(part 1 of 2)
# Autodesk Inventor assembly: Armature
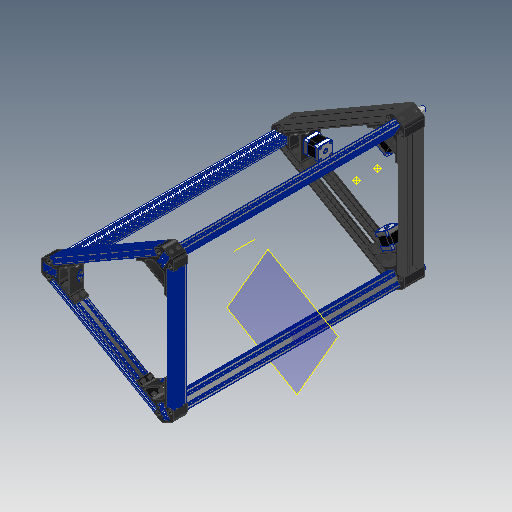
[picture p0: Inventor's stored thumbnail of the model, 512x512]
Saved by Autodesk Inventor 2017 (Build 210142000, 142)
## iProperties
Company: FABLAB Frenchmakers
Part Number: Armature
Material: Générique
Document SubType Name: Assembly
Designer: FABLAB Frenchmakers
Mass: 6567.24 g
Surface Area: 18690.5 cm^2
Volume: 2361.97 cm^3
Density: 2.78041 g/cm^3
Project: 1420 Vauban 3D XL
Stock Number: 1420-01-00
## Documents named in this file (13)
- W:\Professionnel\Conception FABLAB\1420-Vauban 3D XL\1420-01 Armature\1420-01-00 Armature.iam
- W:\Professionnel\Conception FABLAB\1420-Vauban 3D XL\1420-01 Armature\1420-01-14 Coins inferieur.iam
- W:\Professionnel\Conception FABLAB\1420-Vauban 3D XL\1420-01 Armature\1420-01-01 Profile vertical 20x40x750.ipt
- W:\Professionnel\Conception FABLAB\1420-Vauban 3D XL\1420-01 Armature\1420-01-15 Coins superieur.iam
- W:\Professionnel\Conception FABLAB\1420-Vauban 3D XL\1420-01 Armature\1420-01-03 Profile horizontal 20x20x360.ipt
- W:\Professionnel\Conception FABLAB\1420-Vauban 3D XL\1420-01 Armature\1420-01-02 Profile horizontal 20x40x360.ipt
- W:\Professionnel\Conception FABLAB\1420-Vauban 3D XL\1420-90 Centre de contenu\fr-FR\ANSI B18.3.1M(1)\ANSI B18.3.1M - M5x0,8 x 12(2).ipt
- W:\Professionnel\Conception FABLAB\1420-Vauban 3D XL\1420-90 Centre de contenu\fr-FR\DIN 125-1  A\DIN 125 - A 5,3.ipt
- W:\Professionnel\Conception FABLAB\1420-Vauban 3D XL\1420-01 Armature\1420-01-13 Noix M5.ipt
- W:\Professionnel\Conception FABLAB\1420-Vauban 3D XL\1420-90 Centre de contenu\fr-FR\DIN 7991(2)\DIN 7991 - M4x10.ipt
- W:\Professionnel\Conception FABLAB\1420-Vauban 3D XL\1420-01 Armature\1420-01-12 Noix M4.ipt
- W:\Professionnel\Conception FABLAB\1420-Vauban 3D XL\1420-01 Armature\1420-01-09 Pied.ipt
- W:\Professionnel\Conception FABLAB\1420-Vauban 3D XL\1420-90 Centre de contenu\fr-FR\ANSI B18.3.1M(1)\ANSI B18.3.1M - M5x0,8 x 25(2).ipt
## Components (192 placed, 12 different names)
1. 1420-01-09 Pied:1 — Affleurement:196, Placage:246, Placage:247, Placage:250, Placage:251
2. 1420-01-09 Pied:2 — Affleurement:196, Affleurement:197, Placage:249, Placage:253
3. 1420-01-09 Pied:3 — Affleurement:197, Placage:248, Placage:252
4. Vis à tête percée - Métrique M5x0,8 x 25:1 — Affleurement:198, Affleurement:199, Placage:252
5. Vis à tête percée - Métrique M5x0,8 x 25:2 — Affleurement:199, Placage:253
6. Vis à tête percée - Métrique M5x0,8 x 25:3 — Affleurement:198, Placage:250, Placage:251
7. 1420-01-14 Coins inferieur:1 [sub-assembly] — Affleurement:1, Affleurement:2, Affleurement:4, Affleurement:5, Placage:1, Placage:3, Placage:6, Affleurement:8, Placage:12, Placage:13, Affleurement:16, Placage:19, Placage:22, Affleurement:21, Placage:23, Affleurement:22, Placage:28, Placage:43, Placage:44, Placage:45, Placage:46, Placage:51, Placage:52, Placage:53, Placage:54, Placage:65, Placage:66, Placage:67, Placage:68, Placage:69, Placage:71, Placage:72, Placage:73, Placage:74, Placage:75, Placage:214, Placage:215, Placage:245
8. 1420-01-14 Coins inferieur:2 [sub-assembly] — Affleurement:2, Affleurement:3, Affleurement:5, Placage:4, Placage:7, Placage:14, Placage:17, Affleurement:17, Placage:20, Placage:21, Placage:26, Affleurement:25, Placage:27, Affleurement:26, Placage:35, Placage:36, Placage:37, Placage:38, Placage:47, Placage:48, Placage:49, Placage:50, Placage:77, Placage:78, Placage:79, Placage:80, Placage:81, Placage:83, Placage:84, Placage:85, Placage:86, Placage:87, Placage:209, Placage:210, Placage:236
9. 1420-01-14 Coins inferieur:3 [sub-assembly] — Affleurement:1, Affleurement:3, Affleurement:4, Placage:5, Placage:8, Placage:15, Placage:16, Affleurement:15, Symétrie:1, Placage:24, Affleurement:23, Placage:25, Affleurement:24, Placage:39, Placage:40, Placage:41, Placage:42, Placage:55, Placage:56, Placage:57, Placage:58, Placage:59, Placage:60, Placage:61, Placage:62, Placage:63, Placage:89, Placage:90, Placage:91, Placage:92, Placage:93, Placage:216, Placage:217, Placage:239
10. 1420-01-15 Coins superieur:1 [sub-assembly] — Affleurement:10, Affleurement:12, Affleurement:13, Affleurement:14, Affleurement:15, Affleurement:17, Symétrie:1, Affleurement:29, Placage:29, Placage:30, Placage:31, Placage:32, Placage:107, Placage:108, Placage:109, Placage:110, Placage:111, Placage:112, Placage:113, Placage:114, Placage:131, Placage:132, Placage:133, Placage:134, Placage:135, Placage:137, Placage:138, Placage:139, Placage:140, Placage:141, Placage:156, Placage:220, Placage:221, Placage:241
11. 1420-01-15 Coins superieur:2 [sub-assembly] — Affleurement:9, Affleurement:10, Affleurement:11, Affleurement:12, Placage:34, Placage:99, Placage:100, Placage:101, Placage:102, Placage:103, Placage:104, Placage:105, Placage:106, Placage:119, Placage:120, Placage:121, Placage:123, Placage:124, Placage:125, Placage:127, Placage:128, Placage:129, Placage:212, Placage:213, Placage:235
12. 1420-01-15 Coins superieur:3 [sub-assembly] — Affleurement:9, Affleurement:11, Affleurement:13, Affleurement:16, Placage:33, Placage:95, Placage:96, Placage:97, Placage:98, Placage:115, Placage:116, Placage:117, Placage:118, Placage:143, Placage:144, Placage:145, Placage:146, Placage:147, Placage:149, Placage:150, Placage:151, Placage:152, Placage:153, Placage:218, Placage:219, Placage:243
13. 1420-01-02 Profile horizontal 20x40x360:1 — Affleurement:28, Placage:31, Placage:32, Placage:181
14. 1420-01-02 Profile horizontal 20x40x360:2 — Affleurement:27, Affleurement:28, Placage:33, Placage:34, Placage:172
15. 1420-01-02 Profile horizontal 20x40x360:3 — Affleurement:27, Affleurement:29, Placage:29, Placage:30, Placage:159
16. 1420-01-03 Profile horizontal 20x20x360:1 — Affleurement:18, Placage:23, Affleurement:22, Placage:190
17. 1420-01-03 Profile horizontal 20x20x360:2 — Affleurement:18, Placage:19, Placage:22, Affleurement:21
18. 1420-01-03 Profile horizontal 20x20x360:3 — Affleurement:19, Placage:27, Affleurement:26, Placage:28, Placage:208
19. 1420-01-03 Profile horizontal 20x20x360:4 — Affleurement:19, Placage:20, Placage:26, Affleurement:25
20. 1420-01-03 Profile horizontal 20x20x360:5 — Affleurement:20, Placage:21, Placage:24, Affleurement:23, Placage:199
21. 1420-01-03 Profile horizontal 20x20x360:6 — Affleurement:20, Placage:25, Affleurement:24
22. 1420-01-01 Profile vertical 20x40x750:1 — Affleurement:7, Affleurement:8, Placage:12, Placage:13, Placage:242, Placage:244, Placage:249
23. 1420-01-01 Profile vertical 20x40x750:2 — Affleurement:6, Affleurement:7, Placage:14, Placage:17, Placage:234, Placage:237, Placage:246, Placage:247
24. 1420-01-01 Profile vertical 20x40x750:3 — Affleurement:6, Placage:15, Placage:16, Affleurement:14, Placage:238, Placage:240, Placage:248
25. 1420-01-12 Noix M4:8 — Affleurement:193, Placage:233, Affleurement:194, Placage:237
26. 1420-01-12 Noix M4:7 — Affleurement:193, Placage:232, Affleurement:194
27. 1420-01-12 Noix M4:6 — Affleurement:188, Placage:225, Affleurement:189
28. 1420-01-12 Noix M4:5 — Affleurement:188, Placage:224, Affleurement:189, Placage:238
29. 1420-01-12 Noix M4:4 — Affleurement:190, Placage:226
30. 1420-01-12 Noix M4:3 — Affleurement:190, Placage:227, Placage:244
31. 1420-01-13 Noix M5:48 — Affleurement:170, Affleurement:172, Placage:200, Affleurement:175
32. 1420-01-13 Noix M5:47 — Affleurement:171, Affleurement:172, Placage:207, Affleurement:175, Affleurement:176
33. 1420-01-13 Noix M5:46 — Affleurement:171, Placage:206, Affleurement:174, Affleurement:176
34. 1420-01-13 Noix M5:45 — Affleurement:170, Placage:201, Affleurement:173, Placage:208, Affleurement:174
35. 1420-01-13 Noix M5:44 — Affleurement:169, Placage:203, Affleurement:178, Affleurement:179
36. 1420-01-13 Noix M5:43 — Affleurement:167, Placage:204, Affleurement:173, Affleurement:179
37. 1420-01-13 Noix M5:42 — Affleurement:168, Affleurement:169, Placage:202, Affleurement:177, Affleurement:178
38. 1420-01-13 Noix M5:41 — Affleurement:167, Affleurement:168, Placage:205, Affleurement:177
39. 1420-01-13 Noix M5:40 — Affleurement:154, Affleurement:156, Placage:193, Affleurement:161, Affleurement:166
40. 1420-01-13 Noix M5:39 — Affleurement:156, Placage:191, Affleurement:162
41. 1420-01-13 Noix M5:38 — Affleurement:155, Placage:198, Affleurement:160, Affleurement:161
42. 1420-01-13 Noix M5:37 — Affleurement:154, Affleurement:155, Placage:192, Affleurement:160, Affleurement:162
43. 1420-01-13 Noix M5:36 — Affleurement:157, Placage:194, Affleurement:164
44. 1420-01-13 Noix M5:35 — Affleurement:158, Placage:195, Affleurement:163, Affleurement:164
45. 1420-01-13 Noix M5:34 — Affleurement:159, Placage:196, Affleurement:165
46. 1420-01-13 Noix M5:33 — Affleurement:157, Affleurement:158, Affleurement:159, Placage:197, Placage:199, Affleurement:163, Affleurement:165, Affleurement:166
47. 1420-01-13 Noix M5:32 — Affleurement:144, Placage:186, Affleurement:148, Affleurement:149
48. 1420-01-13 Noix M5:31 — Affleurement:145, Affleurement:146, Placage:188, Affleurement:147
49. 1420-01-13 Noix M5:30 — Affleurement:146, Placage:189, Affleurement:147, Affleurement:149, Affleurement:153
50. 1420-01-13 Noix M5:29 — Affleurement:144, Affleurement:145, Placage:187, Affleurement:148
51. 1420-01-13 Noix M5:28 — Affleurement:142, Affleurement:143, Placage:183, Affleurement:151, Affleurement:152, Placage:190
52. 1420-01-13 Noix M5:27 — Affleurement:141, Affleurement:143, Placage:185, Affleurement:150, Affleurement:152, Affleurement:153
53. 1420-01-13 Noix M5:26 — Affleurement:142, Placage:184, Affleurement:150
54. 1420-01-13 Noix M5:25 — Affleurement:141, Placage:182, Affleurement:151
55. DIN 7991 M4x10:1 — Affleurement:180, Placage:209, Placage:233, Placage:236
56. DIN 7991 M4x10:2 — Affleurement:180, Placage:210, Placage:232
57. DIN 7991 M4x10:3 — Affleurement:182, Placage:214, Placage:227
58. DIN 7991 M4x10:4 — Affleurement:182, Placage:215, Placage:226, Placage:245
59. DIN 7991 M4x10:5 — Affleurement:183, Placage:216, Placage:225
60. DIN 7991 M4x10:6 — Affleurement:183, Placage:217, Placage:224, Placage:239
61. Vis à tête percée - Métrique M5x0,8 x 12:1 — Affleurement:30, Placage:42, Placage:94, Placage:195
62. Vis à tête percée - Métrique M5x0,8 x 12:2 — Affleurement:30, Affleurement:31, Placage:41, Placage:196
63. Vis à tête percée - Métrique M5x0,8 x 12:3 — Affleurement:31, Affleurement:32, Placage:39, Placage:197
64. Vis à tête percée - Métrique M5x0,8 x 12:4 — Affleurement:32, Placage:40, Placage:194
65. Vis à tête percée - Métrique M5x0,8 x 12:5 — Affleurement:33, Placage:37, Placage:191
66. Vis à tête percée - Métrique M5x0,8 x 12:6 — Affleurement:33, Affleurement:34, Placage:38, Placage:192
67. Vis à tête percée - Métrique M5x0,8 x 12:7 — Affleurement:34, Affleurement:35, Placage:36, Placage:88, Placage:193
68. Vis à tête percée - Métrique M5x0,8 x 12:8 — Affleurement:35, Placage:35, Placage:198
69. Vis à tête percée - Métrique M5x0,8 x 12:9 — Affleurement:39, Placage:47, Placage:203
70. Vis à tête percée - Métrique M5x0,8 x 12:10 — Affleurement:39, Affleurement:40, Placage:48, Placage:82, Placage:204
71. Vis à tête percée - Métrique M5x0,8 x 12:11 — Affleurement:40, Affleurement:41, Placage:50, Placage:205
72. Vis à tête percée - Métrique M5x0,8 x 12:12 — Affleurement:41, Placage:49, Placage:202
73. Vis à tête percée - Métrique M5x0,8 x 12:13 — Affleurement:36, Placage:43, Placage:201
74. Vis à tête percée - Métrique M5x0,8 x 12:14 — Affleurement:36, Affleurement:37, Placage:44, Placage:76, Placage:206
75. Vis à tête percée - Métrique M5x0,8 x 12:15 — Affleurement:37, Affleurement:38, Placage:45, Placage:200
76. Vis à tête percée - Métrique M5x0,8 x 12:16 — Affleurement:38, Placage:46, Placage:207
77. Vis à tête percée - Métrique M5x0,8 x 12:17 — Placage:56, Affleurement:45, Affleurement:47, Placage:189
78. Vis à tête percée - Métrique M5x0,8 x 12:18 — Placage:57, Affleurement:46, Placage:187
79. Vis à tête percée - Métrique M5x0,8 x 12:19 — Placage:58, Affleurement:47, Placage:186
80. Vis à tête percée - Métrique M5x0,8 x 12:20 — Placage:55, Affleurement:45, Affleurement:46, Placage:64, Placage:188
81. Vis à tête percée - Métrique M5x0,8 x 12:21 — Affleurement:43, Affleurement:44, Placage:52, Placage:70, Placage:184
82. Vis à tête percée - Métrique M5x0,8 x 12:22 — Affleurement:44, Placage:51, Placage:185
83. Vis à tête percée - Métrique M5x0,8 x 12:23 — Affleurement:42, Affleurement:43, Placage:54, Placage:182
84. Vis à tête percée - Métrique M5x0,8 x 12:24 — Affleurement:42, Placage:53, Placage:183
85. DIN 125-1 A A 5,3:1 — Affleurement:50, Placage:59, Placage:60, Placage:64
86. DIN 125-1 A A 5,3:2 — Affleurement:49, Placage:61
87. DIN 125-1 A A 5,3:3 — Affleurement:48, Affleurement:49, Affleurement:50, Placage:63
88. DIN 125-1 A A 5,3:4 — Affleurement:48, Placage:62
89. DIN 125-1 A A 5,3:5 — Affleurement:51, Placage:65, Placage:66, Placage:70
90. DIN 125-1 A A 5,3:6 — Affleurement:51, Affleurement:52, Placage:67
91. DIN 125-1 A A 5,3:7 — Affleurement:52, Affleurement:53, Placage:68
92. DIN 125-1 A A 5,3:8 — Affleurement:53, Placage:69
93. DIN 125-1 A A 5,3:9 — Affleurement:54, Placage:71, Placage:72
94. DIN 125-1 A A 5,3:10 — Affleurement:54, Affleurement:55, Placage:73
95. DIN 125-1 A A 5,3:11 — Affleurement:55, Affleurement:56, Affleurement:57, Placage:75
96. DIN 125-1 A A 5,3:12 — Affleurement:56, Affleurement:57, Placage:74, Placage:76
97. DIN 125-1 A A 5,3:13 — Affleurement:58, Placage:81
98. DIN 125-1 A A 5,3:14 — Affleurement:58, Affleurement:59, Placage:80
99. DIN 125-1 A A 5,3:15 — Affleurement:59, Affleurement:60, Placage:77, Placage:78
100. DIN 125-1 A A 5,3:16 — Affleurement:60, Placage:79, Placage:82
101. DIN 125-1 A A 5,3:17 — Affleurement:63, Placage:86
102. DIN 125-1 A A 5,3:18 — Affleurement:62, Affleurement:63, Placage:85, Placage:88
103. DIN 125-1 A A 5,3:19 — Affleurement:61, Affleurement:62, Placage:83, Placage:84
104. DIN 125-1 A A 5,3:20 — Affleurement:61, Placage:87
105. DIN 125-1 A A 5,3:21 — Affleurement:66, Placage:89, Placage:90
106. DIN 125-1 A A 5,3:22 — Affleurement:65, Affleurement:66, Placage:92
107. DIN 125-1 A A 5,3:23 — Affleurement:64, Affleurement:65, Placage:91, Placage:94
108. DIN 125-1 A A 5,3:24 — Affleurement:64, Placage:93
109. DIN 7991 M4x10:7 — Affleurement:184, Placage:219, Placage:229, Placage:243
110. DIN 7991 M4x10:8 — Affleurement:184, Placage:218, Placage:228
111. DIN 7991 M4x10:9 — Affleurement:185, Placage:220, Placage:223, Placage:241
112. DIN 7991 M4x10:10 — Affleurement:185, Placage:221, Placage:222
113. DIN 7991 M4x10:11 — Affleurement:181, Placage:212, Placage:230, Placage:235
114. DIN 7991 M4x10:12 — Affleurement:181, Placage:213, Placage:231
115. Vis à tête percée - Métrique M5x0,8 x 12:25 — Affleurement:67, Affleurement:68, Placage:97, Placage:170
116. Vis à tête percée - Métrique M5x0,8 x 12:26 — Affleurement:68, Affleurement:69, Placage:96, Placage:169
117. Vis à tête percée - Métrique M5x0,8 x 12:27 — Affleurement:69, Placage:95, Placage:154, Placage:171
118. Vis à tête percée - Métrique M5x0,8 x 12:28 — Affleurement:67, Placage:98, Placage:168
119. Vis à tête percée - Métrique M5x0,8 x 12:29 — Affleurement:70, Placage:99, Placage:122, Placage:166
120. Vis à tête percée - Métrique M5x0,8 x 12:30 — Affleurement:70, Affleurement:71, Placage:100, Placage:126, Placage:167
121. Vis à tête percée - Métrique M5x0,8 x 12:31 — Affleurement:71, Affleurement:72, Placage:101, Placage:165
122. Vis à tête percée - Métrique M5x0,8 x 12:32 — Affleurement:72, Placage:102, Placage:164
123. Vis à tête percée - Métrique M5x0,8 x 12:33 — Affleurement:75, Placage:106, Placage:161
124. Vis à tête percée - Métrique M5x0,8 x 12:34 — Affleurement:74, Affleurement:75, Placage:104, Placage:160
125. Vis à tête percée - Métrique M5x0,8 x 12:35 — Affleurement:73, Affleurement:74, Placage:105, Placage:163
126. Vis à tête percée - Métrique M5x0,8 x 12:36 — Affleurement:73, Placage:103, Placage:130, Placage:162
127. Vis à tête percée - Métrique M5x0,8 x 12:37 — Affleurement:81, Placage:112, Placage:180
128. Vis à tête percée - Métrique M5x0,8 x 12:38 — Affleurement:80, Affleurement:81, Placage:111, Placage:142, Placage:178
129. Vis à tête percée - Métrique M5x0,8 x 12:39 — Affleurement:79, Affleurement:80, Placage:114, Placage:177
130. Vis à tête percée - Métrique M5x0,8 x 12:40 — Affleurement:79, Placage:113, Placage:179
131. Vis à tête percée - Métrique M5x0,8 x 12:41 — Affleurement:77, Affleurement:78, Placage:107
132. Vis à tête percée - Métrique M5x0,8 x 12:42 — Affleurement:76, Affleurement:77, Placage:109, Placage:155
133. Vis à tête percée - Métrique M5x0,8 x 12:43 — Affleurement:76, Placage:108, Placage:158
134. Vis à tête percée - Métrique M5x0,8 x 12:44 — Affleurement:78, Placage:110, Placage:136, Placage:157
135. Vis à tête percée - Métrique M5x0,8 x 12:45 — Affleurement:83, Affleurement:84, Placage:118, Placage:173
136. Vis à tête percée - Métrique M5x0,8 x 12:46 — Affleurement:82, Affleurement:83, Placage:116, Placage:174
137. Vis à tête percée - Métrique M5x0,8 x 12:47 — Affleurement:82, Placage:115, Placage:148, Placage:175
138. Vis à tête percée - Métrique M5x0,8 x 12:49 — Affleurement:84, Placage:117, Placage:176
139. DIN 125-1 A A 5,3:25 — Affleurement:100, Affleurement:101, Affleurement:102, Placage:152
140. DIN 125-1 A A 5,3:26 — Affleurement:102, Placage:153
141. DIN 125-1 A A 5,3:27 — Affleurement:100, Placage:151
142. DIN 125-1 A A 5,3:28 — Affleurement:101, Placage:149, Placage:150, Placage:154
143. DIN 125-1 A A 5,3:29 — Affleurement:99, Placage:146
144. DIN 125-1 A A 5,3:30 — Affleurement:98, Placage:147, Placage:148
145. DIN 125-1 A A 5,3:31 — Affleurement:97, Placage:143, Placage:144
146. DIN 125-1 A A 5,3:32 — Affleurement:97, Affleurement:98, Affleurement:99, Placage:145
147. DIN 125-1 A A 5,3:33 — Affleurement:89, Placage:124
148. DIN 125-1 A A 5,3:34 — Affleurement:88, Affleurement:89, Placage:125
149. DIN 125-1 A A 5,3:35 — Affleurement:88, Affleurement:90, Placage:123, Placage:126
150. DIN 125-1 A A 5,3:36 — Affleurement:90, Placage:121, Placage:122
151. DIN 125-1 A A 5,3:37 — Affleurement:86, Affleurement:87, Placage:128
152. DIN 125-1 A A 5,3:38 — Affleurement:87, Placage:129
153. DIN 125-1 A A 5,3:39 — Affleurement:85, Affleurement:86, Placage:119, Placage:120, Placage:130
154. DIN 125-1 A A 5,3:40 — Affleurement:85, Placage:127
155. DIN 125-1 A A 5,3:41 — Affleurement:91, Placage:131, Placage:132
156. DIN 125-1 A A 5,3:42 — Affleurement:91, Affleurement:92, Affleurement:93, Placage:134
157. DIN 125-1 A A 5,3:43 — Affleurement:92, Placage:133, Placage:136
158. DIN 125-1 A A 5,3:44 — Affleurement:93, Placage:135
159. DIN 125-1 A A 5,3:45 — Affleurement:94, Placage:139
160. DIN 125-1 A A 5,3:46 — Affleurement:94, Affleurement:96, Placage:137, Placage:138
161. DIN 125-1 A A 5,3:47 — Affleurement:95, Placage:141
162. DIN 125-1 A A 5,3:48 — Affleurement:95, Affleurement:96, Placage:140, Placage:142
163. 1420-01-12 Noix M4:1 — Affleurement:191, Placage:228
164. 1420-01-12 Noix M4:2 — Affleurement:191, Placage:229, Placage:242
165. 1420-01-12 Noix M4:9 — Affleurement:186, Placage:223, Affleurement:187, Placage:240
166. 1420-01-12 Noix M4:10 — Affleurement:186, Placage:222, Affleurement:187
167. 1420-01-12 Noix M4:11 — Affleurement:192, Placage:230, Affleurement:195
168. 1420-01-12 Noix M4:12 — Affleurement:192, Placage:231, Affleurement:195, Placage:234
169. 1420-01-13 Noix M5:17 — Affleurement:130, Placage:176, Affleurement:132
170. 1420-01-13 Noix M5:18 — Affleurement:129, Affleurement:130, Affleurement:131, Placage:175, Affleurement:133, Placage:181
171. 1420-01-13 Noix M5:19 — Affleurement:129, Placage:173, Affleurement:132, Affleurement:134, Affleurement:140
172. 1420-01-13 Noix M5:20 — Affleurement:131, Placage:174, Affleurement:133, Affleurement:134
173. 1420-01-13 Noix M5:21 — Affleurement:136, Affleurement:137, Placage:179, Affleurement:139
174. 1420-01-13 Noix M5:22 — Affleurement:135, Placage:177, Affleurement:139, Affleurement:140
175. 1420-01-13 Noix M5:23 — Affleurement:135, Affleurement:136, Placage:178, Affleurement:138
176. 1420-01-13 Noix M5:24 — Affleurement:137, Placage:180, Affleurement:138
177. 1420-01-13 Noix M5:9 — Affleurement:116, Placage:164, Affleurement:126
178. 1420-01-13 Noix M5:10 — Affleurement:116, Affleurement:118, Placage:165, Affleurement:128
179. 1420-01-13 Noix M5:11 — Affleurement:117, Affleurement:118, Placage:166, Placage:172, Affleurement:125, Affleurement:127, Affleurement:128
180. 1420-01-13 Noix M5:12 — Affleurement:117, Placage:167, Affleurement:126, Affleurement:127
181. 1420-01-13 Noix M5:13 — Affleurement:119, Affleurement:120, Placage:168, Affleurement:122
182. 1420-01-13 Noix M5:14 — Affleurement:120, Affleurement:121, Placage:170, Affleurement:124
183. 1420-01-13 Noix M5:15 — Affleurement:121, Placage:171, Affleurement:123, Affleurement:124
184. 1420-01-13 Noix M5:16 — Affleurement:119, Placage:169, Affleurement:122, Affleurement:123, Affleurement:125
185. 1420-01-13 Noix M5:1 — Affleurement:103, Affleurement:104, Placage:156, Affleurement:106, Affleurement:107, Affleurement:112
186. 1420-01-13 Noix M5:2 — Affleurement:103, Placage:158, Placage:159, Affleurement:107, Affleurement:108
187. 1420-01-13 Noix M5:3 — Affleurement:104, Affleurement:105, Placage:155, Affleurement:106
188. 1420-01-13 Noix M5:4 — Affleurement:105, Placage:157, Affleurement:108
189. 1420-01-13 Noix M5:5 — Affleurement:109, Placage:163, Affleurement:114, Affleurement:115
190. 1420-01-13 Noix M5:6 — Affleurement:109, Affleurement:110, Affleurement:111, Placage:160, Affleurement:113
191. 1420-01-13 Noix M5:7 — Affleurement:110, Placage:162, Affleurement:112, Affleurement:115
192. 1420-01-13 Noix M5:8 — Affleurement:111, Placage:161, Affleurement:113, Affleurement:114
## Relationships (451: Mate 251, Flush 199, Symmetry 1)
- Affleurement:1 [Flush]: 1420-01-14 Coins inferieur:1 ↔ 1420-01-14 Coins inferieur:3
- Affleurement:2 [Flush]: 1420-01-14 Coins inferieur:1 ↔ 1420-01-14 Coins inferieur:2
- Affleurement:3 [Flush]: 1420-01-14 Coins inferieur:2 ↔ 1420-01-14 Coins inferieur:3
- Affleurement:4 [Flush]: 1420-01-14 Coins inferieur:1 ↔ 1420-01-14 Coins inferieur:3
- Affleurement:5 [Flush]: 1420-01-14 Coins inferieur:1 ↔ 1420-01-14 Coins inferieur:2
- Placage:1 [Mate]: 1420-01-14 Coins inferieur:1
- Placage:3 [Mate]: 1420-01-14 Coins inferieur:1
- Placage:4 [Mate]: 1420-01-14 Coins inferieur:2
- Placage:5 [Mate]: 1420-01-14 Coins inferieur:3
- Placage:6 [Mate]: 1420-01-14 Coins inferieur:1
- Placage:7 [Mate]: 1420-01-14 Coins inferieur:2
- Placage:8 [Mate]: 1420-01-14 Coins inferieur:3
- Placage:9 [Mate]
- Placage:10 [Mate]
- Placage:11 [Mate]
- Affleurement:6 [Flush]: 1420-01-01 Profile vertical 20x40x750:2 ↔ 1420-01-01 Profile vertical 20x40x750:3
- Affleurement:7 [Flush]: 1420-01-01 Profile vertical 20x40x750:1 ↔ 1420-01-01 Profile vertical 20x40x750:2
- Affleurement:8 [Flush]: 1420-01-14 Coins inferieur:1 ↔ 1420-01-01 Profile vertical 20x40x750:1
- Placage:12 [Mate]: 1420-01-14 Coins inferieur:1 ↔ 1420-01-01 Profile vertical 20x40x750:1
- Placage:13 [Mate]: 1420-01-14 Coins inferieur:1 ↔ 1420-01-01 Profile vertical 20x40x750:1
- Placage:14 [Mate]: 1420-01-14 Coins inferieur:2 ↔ 1420-01-01 Profile vertical 20x40x750:2
- Placage:15 [Mate]: 1420-01-14 Coins inferieur:3 ↔ 1420-01-01 Profile vertical 20x40x750:3
- Placage:16 [Mate]: 1420-01-14 Coins inferieur:3 ↔ 1420-01-01 Profile vertical 20x40x750:3
- Placage:17 [Mate]: 1420-01-14 Coins inferieur:2 ↔ 1420-01-01 Profile vertical 20x40x750:2
- Affleurement:9 [Flush]: 1420-01-15 Coins superieur:2 ↔ 1420-01-15 Coins superieur:3
- Affleurement:10 [Flush]: 1420-01-15 Coins superieur:1 ↔ 1420-01-15 Coins superieur:2
- Affleurement:11 [Flush]: 1420-01-15 Coins superieur:2 ↔ 1420-01-15 Coins superieur:3
- Affleurement:12 [Flush]: 1420-01-15 Coins superieur:1 ↔ 1420-01-15 Coins superieur:2
- Affleurement:13 [Flush]: 1420-01-15 Coins superieur:1 ↔ 1420-01-15 Coins superieur:3
- Affleurement:14 [Flush]: 1420-01-15 Coins superieur:1 ↔ 1420-01-01 Profile vertical 20x40x750:3
- Affleurement:15 [Flush]: 1420-01-14 Coins inferieur:3 ↔ 1420-01-15 Coins superieur:1
- Affleurement:16 [Flush]: 1420-01-14 Coins inferieur:1 ↔ 1420-01-15 Coins superieur:3
- Affleurement:17 [Flush]: 1420-01-14 Coins inferieur:2 ↔ 1420-01-15 Coins superieur:1
- Symétrie:1 [Symmetry]: 1420-01-14 Coins inferieur:3 ↔ 1420-01-15 Coins superieur:1
- Placage:18 [Mate]
- Affleurement:18 [Flush]: 1420-01-03 Profile horizontal 20x20x360:1 ↔ 1420-01-03 Profile horizontal 20x20x360:2
- Affleurement:19 [Flush]: 1420-01-03 Profile horizontal 20x20x360:3 ↔ 1420-01-03 Profile horizontal 20x20x360:4
- Affleurement:20 [Flush]: 1420-01-03 Profile horizontal 20x20x360:5 ↔ 1420-01-03 Profile horizontal 20x20x360:6
- Placage:19 [Mate]: 1420-01-14 Coins inferieur:1 ↔ 1420-01-03 Profile horizontal 20x20x360:2
- Placage:20 [Mate]: 1420-01-14 Coins inferieur:2 ↔ 1420-01-03 Profile horizontal 20x20x360:4
- Placage:21 [Mate]: 1420-01-14 Coins inferieur:2 ↔ 1420-01-03 Profile horizontal 20x20x360:5
- Placage:22 [Mate]: 1420-01-14 Coins inferieur:1 ↔ 1420-01-03 Profile horizontal 20x20x360:2
- Affleurement:21 [Flush]: 1420-01-14 Coins inferieur:1 ↔ 1420-01-03 Profile horizontal 20x20x360:2
- Placage:23 [Mate]: 1420-01-14 Coins inferieur:1 ↔ 1420-01-03 Profile horizontal 20x20x360:1
- Affleurement:22 [Flush]: 1420-01-14 Coins inferieur:1 ↔ 1420-01-03 Profile horizontal 20x20x360:1
- Placage:24 [Mate]: 1420-01-14 Coins inferieur:3 ↔ 1420-01-03 Profile horizontal 20x20x360:5
- Affleurement:23 [Flush]: 1420-01-14 Coins inferieur:3 ↔ 1420-01-03 Profile horizontal 20x20x360:5
- Placage:25 [Mate]: 1420-01-14 Coins inferieur:3 ↔ 1420-01-03 Profile horizontal 20x20x360:6
- Affleurement:24 [Flush]: 1420-01-14 Coins inferieur:3 ↔ 1420-01-03 Profile horizontal 20x20x360:6
- Placage:26 [Mate]: 1420-01-14 Coins inferieur:2 ↔ 1420-01-03 Profile horizontal 20x20x360:4
- Affleurement:25 [Flush]: 1420-01-14 Coins inferieur:2 ↔ 1420-01-03 Profile horizontal 20x20x360:4
- Placage:27 [Mate]: 1420-01-14 Coins inferieur:2 ↔ 1420-01-03 Profile horizontal 20x20x360:3
- Affleurement:26 [Flush]: 1420-01-14 Coins inferieur:2 ↔ 1420-01-03 Profile horizontal 20x20x360:3
- Placage:28 [Mate]: 1420-01-14 Coins inferieur:1 ↔ 1420-01-03 Profile horizontal 20x20x360:3
- Affleurement:27 [Flush]: 1420-01-02 Profile horizontal 20x40x360:2 ↔ 1420-01-02 Profile horizontal 20x40x360:3
- Affleurement:28 [Flush]: 1420-01-02 Profile horizontal 20x40x360:1 ↔ 1420-01-02 Profile horizontal 20x40x360:2
- Affleurement:29 [Flush]: 1420-01-15 Coins superieur:1 ↔ 1420-01-02 Profile horizontal 20x40x360:3
- Placage:29 [Mate]: 1420-01-15 Coins superieur:1 ↔ 1420-01-02 Profile horizontal 20x40x360:3
- Placage:30 [Mate]: 1420-01-15 Coins superieur:1 ↔ 1420-01-02 Profile horizontal 20x40x360:3
- Placage:31 [Mate]: 1420-01-15 Coins superieur:1 ↔ 1420-01-02 Profile horizontal 20x40x360:1
- Placage:32 [Mate]: 1420-01-15 Coins superieur:1 ↔ 1420-01-02 Profile horizontal 20x40x360:1
- Placage:33 [Mate]: 1420-01-15 Coins superieur:3 ↔ 1420-01-02 Profile horizontal 20x40x360:2
- Placage:34 [Mate]: 1420-01-15 Coins superieur:2 ↔ 1420-01-02 Profile horizontal 20x40x360:2
- Affleurement:30 [Flush]: Vis à tête percée - Métrique M5x0,8 x 12:1 ↔ Vis à tête percée - Métrique M5x0,8 x 12:2
- Affleurement:31 [Flush]: Vis à tête percée - Métrique M5x0,8 x 12:2 ↔ Vis à tête percée - Métrique M5x0,8 x 12:3
- Affleurement:32 [Flush]: Vis à tête percée - Métrique M5x0,8 x 12:3 ↔ Vis à tête percée - Métrique M5x0,8 x 12:4
- Affleurement:33 [Flush]: Vis à tête percée - Métrique M5x0,8 x 12:5 ↔ Vis à tête percée - Métrique M5x0,8 x 12:6
- Affleurement:34 [Flush]: Vis à tête percée - Métrique M5x0,8 x 12:6 ↔ Vis à tête percée - Métrique M5x0,8 x 12:7
- Affleurement:35 [Flush]: Vis à tête percée - Métrique M5x0,8 x 12:7 ↔ Vis à tête percée - Métrique M5x0,8 x 12:8
- Placage:35 [Mate]: 1420-01-14 Coins inferieur:2 ↔ Vis à tête percée - Métrique M5x0,8 x 12:8
- Placage:36 [Mate]: 1420-01-14 Coins inferieur:2 ↔ Vis à tête percée - Métrique M5x0,8 x 12:7
- Placage:37 [Mate]: 1420-01-14 Coins inferieur:2 ↔ Vis à tête percée - Métrique M5x0,8 x 12:5
- Placage:38 [Mate]: 1420-01-14 Coins inferieur:2 ↔ Vis à tête percée - Métrique M5x0,8 x 12:6
- Placage:39 [Mate]: 1420-01-14 Coins inferieur:3 ↔ Vis à tête percée - Métrique M5x0,8 x 12:3
- Placage:40 [Mate]: 1420-01-14 Coins inferieur:3 ↔ Vis à tête percée - Métrique M5x0,8 x 12:4
- Placage:41 [Mate]: 1420-01-14 Coins inferieur:3 ↔ Vis à tête percée - Métrique M5x0,8 x 12:2
- Placage:42 [Mate]: 1420-01-14 Coins inferieur:3 ↔ Vis à tête percée - Métrique M5x0,8 x 12:1
- Affleurement:36 [Flush]: Vis à tête percée - Métrique M5x0,8 x 12:13 ↔ Vis à tête percée - Métrique M5x0,8 x 12:14
- Affleurement:37 [Flush]: Vis à tête percée - Métrique M5x0,8 x 12:14 ↔ Vis à tête percée - Métrique M5x0,8 x 12:15
- Affleurement:38 [Flush]: Vis à tête percée - Métrique M5x0,8 x 12:15 ↔ Vis à tête percée - Métrique M5x0,8 x 12:16
- Affleurement:39 [Flush]: Vis à tête percée - Métrique M5x0,8 x 12:9 ↔ Vis à tête percée - Métrique M5x0,8 x 12:10
- Affleurement:40 [Flush]: Vis à tête percée - Métrique M5x0,8 x 12:10 ↔ Vis à tête percée - Métrique M5x0,8 x 12:11
- Affleurement:41 [Flush]: Vis à tête percée - Métrique M5x0,8 x 12:11 ↔ Vis à tête percée - Métrique M5x0,8 x 12:12
- Placage:43 [Mate]: 1420-01-14 Coins inferieur:1 ↔ Vis à tête percée - Métrique M5x0,8 x 12:13
- Placage:44 [Mate]: 1420-01-14 Coins inferieur:1 ↔ Vis à tête percée - Métrique M5x0,8 x 12:14
- Placage:45 [Mate]: 1420-01-14 Coins inferieur:1 ↔ Vis à tête percée - Métrique M5x0,8 x 12:15
- Placage:46 [Mate]: 1420-01-14 Coins inferieur:1 ↔ Vis à tête percée - Métrique M5x0,8 x 12:16
- Placage:47 [Mate]: 1420-01-14 Coins inferieur:2 ↔ Vis à tête percée - Métrique M5x0,8 x 12:9
- Placage:48 [Mate]: 1420-01-14 Coins inferieur:2 ↔ Vis à tête percée - Métrique M5x0,8 x 12:10
- Placage:49 [Mate]: 1420-01-14 Coins inferieur:2 ↔ Vis à tête percée - Métrique M5x0,8 x 12:12
- Placage:50 [Mate]: 1420-01-14 Coins inferieur:2 ↔ Vis à tête percée - Métrique M5x0,8 x 12:11
- Affleurement:42 [Flush]: Vis à tête percée - Métrique M5x0,8 x 12:23 ↔ Vis à tête percée - Métrique M5x0,8 x 12:24
- Affleurement:43 [Flush]: Vis à tête percée - Métrique M5x0,8 x 12:21 ↔ Vis à tête percée - Métrique M5x0,8 x 12:23
- Affleurement:44 [Flush]: Vis à tête percée - Métrique M5x0,8 x 12:21 ↔ Vis à tête percée - Métrique M5x0,8 x 12:22
- Placage:51 [Mate]: 1420-01-14 Coins inferieur:1 ↔ Vis à tête percée - Métrique M5x0,8 x 12:22
- Placage:52 [Mate]: 1420-01-14 Coins inferieur:1 ↔ Vis à tête percée - Métrique M5x0,8 x 12:21
- Placage:53 [Mate]: 1420-01-14 Coins inferieur:1 ↔ Vis à tête percée - Métrique M5x0,8 x 12:24
- Placage:54 [Mate]: 1420-01-14 Coins inferieur:1 ↔ Vis à tête percée - Métrique M5x0,8 x 12:23
- Placage:55 [Mate]: 1420-01-14 Coins inferieur:3 ↔ Vis à tête percée - Métrique M5x0,8 x 12:20
- Placage:56 [Mate]: 1420-01-14 Coins inferieur:3 ↔ Vis à tête percée - Métrique M5x0,8 x 12:17
- Placage:57 [Mate]: 1420-01-14 Coins inferieur:3 ↔ Vis à tête percée - Métrique M5x0,8 x 12:18
- Placage:58 [Mate]: 1420-01-14 Coins inferieur:3 ↔ Vis à tête percée - Métrique M5x0,8 x 12:19
- Affleurement:45 [Flush]: Vis à tête percée - Métrique M5x0,8 x 12:17 ↔ Vis à tête percée - Métrique M5x0,8 x 12:20
- Affleurement:46 [Flush]: Vis à tête percée - Métrique M5x0,8 x 12:18 ↔ Vis à tête percée - Métrique M5x0,8 x 12:20
- Affleurement:47 [Flush]: Vis à tête percée - Métrique M5x0,8 x 12:17 ↔ Vis à tête percée - Métrique M5x0,8 x 12:19
- Affleurement:48 [Flush]: DIN 125-1 A A 5,3:3 ↔ DIN 125-1 A A 5,3:4
- Affleurement:49 [Flush]: DIN 125-1 A A 5,3:2 ↔ DIN 125-1 A A 5,3:3
- Affleurement:50 [Flush]: DIN 125-1 A A 5,3:1 ↔ DIN 125-1 A A 5,3:3
- Affleurement:51 [Flush]: DIN 125-1 A A 5,3:5 ↔ DIN 125-1 A A 5,3:6
- Affleurement:52 [Flush]: DIN 125-1 A A 5,3:6 ↔ DIN 125-1 A A 5,3:7
- Affleurement:53 [Flush]: DIN 125-1 A A 5,3:7 ↔ DIN 125-1 A A 5,3:8
- Affleurement:54 [Flush]: DIN 125-1 A A 5,3:9 ↔ DIN 125-1 A A 5,3:10
- Affleurement:55 [Flush]: DIN 125-1 A A 5,3:10 ↔ DIN 125-1 A A 5,3:11
- Affleurement:56 [Flush]: DIN 125-1 A A 5,3:11 ↔ DIN 125-1 A A 5,3:12
- Affleurement:57 [Flush]: DIN 125-1 A A 5,3:11 ↔ DIN 125-1 A A 5,3:12
- Affleurement:58 [Flush]: DIN 125-1 A A 5,3:13 ↔ DIN 125-1 A A 5,3:14
- Affleurement:59 [Flush]: DIN 125-1 A A 5,3:14 ↔ DIN 125-1 A A 5,3:15
- Affleurement:60 [Flush]: DIN 125-1 A A 5,3:15 ↔ DIN 125-1 A A 5,3:16
- Affleurement:61 [Flush]: DIN 125-1 A A 5,3:19 ↔ DIN 125-1 A A 5,3:20
- Affleurement:62 [Flush]: DIN 125-1 A A 5,3:18 ↔ DIN 125-1 A A 5,3:19
- Affleurement:63 [Flush]: DIN 125-1 A A 5,3:17 ↔ DIN 125-1 A A 5,3:18
- Affleurement:64 [Flush]: DIN 125-1 A A 5,3:23 ↔ DIN 125-1 A A 5,3:24
- Affleurement:65 [Flush]: DIN 125-1 A A 5,3:22 ↔ DIN 125-1 A A 5,3:23
- Affleurement:66 [Flush]: DIN 125-1 A A 5,3:21 ↔ DIN 125-1 A A 5,3:22
- Placage:59 [Mate]: 1420-01-14 Coins inferieur:3 ↔ DIN 125-1 A A 5,3:1
- Placage:60 [Mate]: 1420-01-14 Coins inferieur:3 ↔ DIN 125-1 A A 5,3:1
- Placage:61 [Mate]: 1420-01-14 Coins inferieur:3 ↔ DIN 125-1 A A 5,3:2
- Placage:62 [Mate]: 1420-01-14 Coins inferieur:3 ↔ DIN 125-1 A A 5,3:4
- Placage:63 [Mate]: 1420-01-14 Coins inferieur:3 ↔ DIN 125-1 A A 5,3:3
- Placage:64 [Mate]: Vis à tête percée - Métrique M5x0,8 x 12:20 ↔ DIN 125-1 A A 5,3:1
- Placage:65 [Mate]: 1420-01-14 Coins inferieur:1 ↔ DIN 125-1 A A 5,3:5
- Placage:66 [Mate]: 1420-01-14 Coins inferieur:1 ↔ DIN 125-1 A A 5,3:5
- Placage:67 [Mate]: 1420-01-14 Coins inferieur:1 ↔ DIN 125-1 A A 5,3:6
- Placage:68 [Mate]: 1420-01-14 Coins inferieur:1 ↔ DIN 125-1 A A 5,3:7
- Placage:69 [Mate]: 1420-01-14 Coins inferieur:1 ↔ DIN 125-1 A A 5,3:8
- Placage:70 [Mate]: Vis à tête percée - Métrique M5x0,8 x 12:21 ↔ DIN 125-1 A A 5,3:5
- Placage:71 [Mate]: 1420-01-14 Coins inferieur:1 ↔ DIN 125-1 A A 5,3:9
- Placage:72 [Mate]: 1420-01-14 Coins inferieur:1 ↔ DIN 125-1 A A 5,3:9
- Placage:73 [Mate]: 1420-01-14 Coins inferieur:1 ↔ DIN 125-1 A A 5,3:10
- Placage:74 [Mate]: 1420-01-14 Coins inferieur:1 ↔ DIN 125-1 A A 5,3:12
- Placage:75 [Mate]: 1420-01-14 Coins inferieur:1 ↔ DIN 125-1 A A 5,3:11
- Placage:76 [Mate]: Vis à tête percée - Métrique M5x0,8 x 12:14 ↔ DIN 125-1 A A 5,3:12
- Placage:77 [Mate]: 1420-01-14 Coins inferieur:2 ↔ DIN 125-1 A A 5,3:15
- Placage:78 [Mate]: 1420-01-14 Coins inferieur:2 ↔ DIN 125-1 A A 5,3:15
- Placage:79 [Mate]: 1420-01-14 Coins inferieur:2 ↔ DIN 125-1 A A 5,3:16
- Placage:80 [Mate]: 1420-01-14 Coins inferieur:2 ↔ DIN 125-1 A A 5,3:14
- Placage:81 [Mate]: 1420-01-14 Coins inferieur:2 ↔ DIN 125-1 A A 5,3:13
- Placage:82 [Mate]: Vis à tête percée - Métrique M5x0,8 x 12:10 ↔ DIN 125-1 A A 5,3:16
- Placage:83 [Mate]: 1420-01-14 Coins inferieur:2 ↔ DIN 125-1 A A 5,3:19
- Placage:84 [Mate]: 1420-01-14 Coins inferieur:2 ↔ DIN 125-1 A A 5,3:19
- Placage:85 [Mate]: 1420-01-14 Coins inferieur:2 ↔ DIN 125-1 A A 5,3:18
- Placage:86 [Mate]: 1420-01-14 Coins inferieur:2 ↔ DIN 125-1 A A 5,3:17
- Placage:87 [Mate]: 1420-01-14 Coins inferieur:2 ↔ DIN 125-1 A A 5,3:20
- Placage:88 [Mate]: Vis à tête percée - Métrique M5x0,8 x 12:7 ↔ DIN 125-1 A A 5,3:18
- Placage:89 [Mate]: 1420-01-14 Coins inferieur:3 ↔ DIN 125-1 A A 5,3:21
- Placage:90 [Mate]: 1420-01-14 Coins inferieur:3 ↔ DIN 125-1 A A 5,3:21
- Placage:91 [Mate]: 1420-01-14 Coins inferieur:3 ↔ DIN 125-1 A A 5,3:23
- Placage:92 [Mate]: 1420-01-14 Coins inferieur:3 ↔ DIN 125-1 A A 5,3:22
- Placage:93 [Mate]: 1420-01-14 Coins inferieur:3 ↔ DIN 125-1 A A 5,3:24
- Placage:94 [Mate]: Vis à tête percée - Métrique M5x0,8 x 12:1 ↔ DIN 125-1 A A 5,3:23
- Affleurement:67 [Flush]: Vis à tête percée - Métrique M5x0,8 x 12:25 ↔ Vis à tête percée - Métrique M5x0,8 x 12:28
- Affleurement:68 [Flush]: Vis à tête percée - Métrique M5x0,8 x 12:25 ↔ Vis à tête percée - Métrique M5x0,8 x 12:26
- Affleurement:69 [Flush]: Vis à tête percée - Métrique M5x0,8 x 12:26 ↔ Vis à tête percée - Métrique M5x0,8 x 12:27
- Placage:95 [Mate]: 1420-01-15 Coins superieur:3 ↔ Vis à tête percée - Métrique M5x0,8 x 12:27
- Placage:96 [Mate]: 1420-01-15 Coins superieur:3 ↔ Vis à tête percée - Métrique M5x0,8 x 12:26
- Placage:97 [Mate]: 1420-01-15 Coins superieur:3 ↔ Vis à tête percée - Métrique M5x0,8 x 12:25
- Placage:98 [Mate]: 1420-01-15 Coins superieur:3 ↔ Vis à tête percée - Métrique M5x0,8 x 12:28
- Affleurement:70 [Flush]: Vis à tête percée - Métrique M5x0,8 x 12:29 ↔ Vis à tête percée - Métrique M5x0,8 x 12:30
- Affleurement:71 [Flush]: Vis à tête percée - Métrique M5x0,8 x 12:30 ↔ Vis à tête percée - Métrique M5x0,8 x 12:31
- Affleurement:72 [Flush]: Vis à tête percée - Métrique M5x0,8 x 12:31 ↔ Vis à tête percée - Métrique M5x0,8 x 12:32
- Placage:99 [Mate]: 1420-01-15 Coins superieur:2 ↔ Vis à tête percée - Métrique M5x0,8 x 12:29
- Placage:100 [Mate]: 1420-01-15 Coins superieur:2 ↔ Vis à tête percée - Métrique M5x0,8 x 12:30
- Placage:101 [Mate]: 1420-01-15 Coins superieur:2 ↔ Vis à tête percée - Métrique M5x0,8 x 12:31
- Placage:102 [Mate]: 1420-01-15 Coins superieur:2 ↔ Vis à tête percée - Métrique M5x0,8 x 12:32
- Affleurement:73 [Flush]: Vis à tête percée - Métrique M5x0,8 x 12:35 ↔ Vis à tête percée - Métrique M5x0,8 x 12:36
- Affleurement:74 [Flush]: Vis à tête percée - Métrique M5x0,8 x 12:34 ↔ Vis à tête percée - Métrique M5x0,8 x 12:35
- Affleurement:75 [Flush]: Vis à tête percée - Métrique M5x0,8 x 12:33 ↔ Vis à tête percée - Métrique M5x0,8 x 12:34
- Placage:103 [Mate]: 1420-01-15 Coins superieur:2 ↔ Vis à tête percée - Métrique M5x0,8 x 12:36
- Placage:104 [Mate]: 1420-01-15 Coins superieur:2 ↔ Vis à tête percée - Métrique M5x0,8 x 12:34
- Placage:105 [Mate]: 1420-01-15 Coins superieur:2 ↔ Vis à tête percée - Métrique M5x0,8 x 12:35
- Placage:106 [Mate]: 1420-01-15 Coins superieur:2 ↔ Vis à tête percée - Métrique M5x0,8 x 12:33
- Affleurement:76 [Flush]: Vis à tête percée - Métrique M5x0,8 x 12:42 ↔ Vis à tête percée - Métrique M5x0,8 x 12:43
- Affleurement:77 [Flush]: Vis à tête percée - Métrique M5x0,8 x 12:41 ↔ Vis à tête percée - Métrique M5x0,8 x 12:42
- Affleurement:78 [Flush]: Vis à tête percée - Métrique M5x0,8 x 12:41 ↔ Vis à tête percée - Métrique M5x0,8 x 12:44
- Placage:107 [Mate]: 1420-01-15 Coins superieur:1 ↔ Vis à tête percée - Métrique M5x0,8 x 12:41
- Placage:108 [Mate]: 1420-01-15 Coins superieur:1 ↔ Vis à tête percée - Métrique M5x0,8 x 12:43
- Placage:109 [Mate]: 1420-01-15 Coins superieur:1 ↔ Vis à tête percée - Métrique M5x0,8 x 12:42
- Placage:110 [Mate]: 1420-01-15 Coins superieur:1 ↔ Vis à tête percée - Métrique M5x0,8 x 12:44
- Affleurement:79 [Flush]: Vis à tête percée - Métrique M5x0,8 x 12:39 ↔ Vis à tête percée - Métrique M5x0,8 x 12:40
- Affleurement:80 [Flush]: Vis à tête percée - Métrique M5x0,8 x 12:38 ↔ Vis à tête percée - Métrique M5x0,8 x 12:39
- Affleurement:81 [Flush]: Vis à tête percée - Métrique M5x0,8 x 12:37 ↔ Vis à tête percée - Métrique M5x0,8 x 12:38
- Placage:111 [Mate]: 1420-01-15 Coins superieur:1 ↔ Vis à tête percée - Métrique M5x0,8 x 12:38
- Placage:112 [Mate]: 1420-01-15 Coins superieur:1 ↔ Vis à tête percée - Métrique M5x0,8 x 12:37
- Placage:113 [Mate]: 1420-01-15 Coins superieur:1 ↔ Vis à tête percée - Métrique M5x0,8 x 12:40
- Placage:114 [Mate]: 1420-01-15 Coins superieur:1 ↔ Vis à tête percée - Métrique M5x0,8 x 12:39
- Affleurement:82 [Flush]: Vis à tête percée - Métrique M5x0,8 x 12:46 ↔ Vis à tête percée - Métrique M5x0,8 x 12:47
- Affleurement:83 [Flush]: Vis à tête percée - Métrique M5x0,8 x 12:45 ↔ Vis à tête percée - Métrique M5x0,8 x 12:46
- Affleurement:84 [Flush]: Vis à tête percée - Métrique M5x0,8 x 12:45 ↔ Vis à tête percée - Métrique M5x0,8 x 12:49
- Placage:115 [Mate]: 1420-01-15 Coins superieur:3 ↔ Vis à tête percée - Métrique M5x0,8 x 12:47
- Placage:116 [Mate]: 1420-01-15 Coins superieur:3 ↔ Vis à tête percée - Métrique M5x0,8 x 12:46
- Placage:117 [Mate]: 1420-01-15 Coins superieur:3 ↔ Vis à tête percée - Métrique M5x0,8 x 12:49
- Placage:118 [Mate]: 1420-01-15 Coins superieur:3 ↔ Vis à tête percée - Métrique M5x0,8 x 12:45
- Affleurement:85 [Flush]: DIN 125-1 A A 5,3:39 ↔ DIN 125-1 A A 5,3:40
- Affleurement:86 [Flush]: DIN 125-1 A A 5,3:37 ↔ DIN 125-1 A A 5,3:39
- Affleurement:87 [Flush]: DIN 125-1 A A 5,3:37 ↔ DIN 125-1 A A 5,3:38
- Placage:119 [Mate]: 1420-01-15 Coins superieur:2 ↔ DIN 125-1 A A 5,3:39
- Placage:120 [Mate]: 1420-01-15 Coins superieur:2 ↔ DIN 125-1 A A 5,3:39
- Affleurement:88 [Flush]: DIN 125-1 A A 5,3:34 ↔ DIN 125-1 A A 5,3:35
- Affleurement:89 [Flush]: DIN 125-1 A A 5,3:33 ↔ DIN 125-1 A A 5,3:34
- Affleurement:90 [Flush]: DIN 125-1 A A 5,3:35 ↔ DIN 125-1 A A 5,3:36
- Placage:121 [Mate]: 1420-01-15 Coins superieur:2 ↔ DIN 125-1 A A 5,3:36
- Placage:122 [Mate]: Vis à tête percée - Métrique M5x0,8 x 12:29 ↔ DIN 125-1 A A 5,3:36
- Placage:123 [Mate]: 1420-01-15 Coins superieur:2 ↔ DIN 125-1 A A 5,3:35
- Placage:124 [Mate]: 1420-01-15 Coins superieur:2 ↔ DIN 125-1 A A 5,3:33
- Placage:125 [Mate]: 1420-01-15 Coins superieur:2 ↔ DIN 125-1 A A 5,3:34
- Placage:126 [Mate]: Vis à tête percée - Métrique M5x0,8 x 12:30 ↔ DIN 125-1 A A 5,3:35
- Placage:127 [Mate]: 1420-01-15 Coins superieur:2 ↔ DIN 125-1 A A 5,3:40
- Placage:128 [Mate]: 1420-01-15 Coins superieur:2 ↔ DIN 125-1 A A 5,3:37
- Placage:129 [Mate]: 1420-01-15 Coins superieur:2 ↔ DIN 125-1 A A 5,3:38
- Placage:130 [Mate]: Vis à tête percée - Métrique M5x0,8 x 12:36 ↔ DIN 125-1 A A 5,3:39
- Affleurement:91 [Flush]: DIN 125-1 A A 5,3:41 ↔ DIN 125-1 A A 5,3:42
- Affleurement:92 [Flush]: DIN 125-1 A A 5,3:42 ↔ DIN 125-1 A A 5,3:43
- Affleurement:93 [Flush]: DIN 125-1 A A 5,3:42 ↔ DIN 125-1 A A 5,3:44
- Placage:131 [Mate]: 1420-01-15 Coins superieur:1 ↔ DIN 125-1 A A 5,3:41
- Placage:132 [Mate]: 1420-01-15 Coins superieur:1 ↔ DIN 125-1 A A 5,3:41
- Placage:133 [Mate]: 1420-01-15 Coins superieur:1 ↔ DIN 125-1 A A 5,3:43
- Placage:134 [Mate]: 1420-01-15 Coins superieur:1 ↔ DIN 125-1 A A 5,3:42
- Placage:135 [Mate]: 1420-01-15 Coins superieur:1 ↔ DIN 125-1 A A 5,3:44
- Placage:136 [Mate]: Vis à tête percée - Métrique M5x0,8 x 12:44 ↔ DIN 125-1 A A 5,3:43
- Affleurement:94 [Flush]: DIN 125-1 A A 5,3:45 ↔ DIN 125-1 A A 5,3:46
- Affleurement:95 [Flush]: DIN 125-1 A A 5,3:47 ↔ DIN 125-1 A A 5,3:48
- Affleurement:96 [Flush]: DIN 125-1 A A 5,3:46 ↔ DIN 125-1 A A 5,3:48
- Placage:137 [Mate]: 1420-01-15 Coins superieur:1 ↔ DIN 125-1 A A 5,3:46
- Placage:138 [Mate]: 1420-01-15 Coins superieur:1 ↔ DIN 125-1 A A 5,3:46
- Placage:139 [Mate]: 1420-01-15 Coins superieur:1 ↔ DIN 125-1 A A 5,3:45
- Placage:140 [Mate]: 1420-01-15 Coins superieur:1 ↔ DIN 125-1 A A 5,3:48
- Placage:141 [Mate]: 1420-01-15 Coins superieur:1 ↔ DIN 125-1 A A 5,3:47
- Placage:142 [Mate]: Vis à tête percée - Métrique M5x0,8 x 12:38 ↔ DIN 125-1 A A 5,3:48
- Affleurement:97 [Flush]: DIN 125-1 A A 5,3:31 ↔ DIN 125-1 A A 5,3:32
- Affleurement:98 [Flush]: DIN 125-1 A A 5,3:30 ↔ DIN 125-1 A A 5,3:32
- Affleurement:99 [Flush]: DIN 125-1 A A 5,3:29 ↔ DIN 125-1 A A 5,3:32
- Placage:143 [Mate]: 1420-01-15 Coins superieur:3 ↔ DIN 125-1 A A 5,3:31
- Placage:144 [Mate]: 1420-01-15 Coins superieur:3 ↔ DIN 125-1 A A 5,3:31
- Placage:145 [Mate]: 1420-01-15 Coins superieur:3 ↔ DIN 125-1 A A 5,3:32
- Placage:146 [Mate]: 1420-01-15 Coins superieur:3 ↔ DIN 125-1 A A 5,3:29
- Placage:147 [Mate]: 1420-01-15 Coins superieur:3 ↔ DIN 125-1 A A 5,3:30
- Placage:148 [Mate]: Vis à tête percée - Métrique M5x0,8 x 12:47 ↔ DIN 125-1 A A 5,3:30
- Affleurement:100 [Flush]: DIN 125-1 A A 5,3:25 ↔ DIN 125-1 A A 5,3:27
- Affleurement:101 [Flush]: DIN 125-1 A A 5,3:25 ↔ DIN 125-1 A A 5,3:28
- Affleurement:102 [Flush]: DIN 125-1 A A 5,3:25 ↔ DIN 125-1 A A 5,3:26
- Placage:149 [Mate]: 1420-01-15 Coins superieur:3 ↔ DIN 125-1 A A 5,3:28
- Placage:150 [Mate]: 1420-01-15 Coins superieur:3 ↔ DIN 125-1 A A 5,3:28
- Placage:151 [Mate]: 1420-01-15 Coins superieur:3 ↔ DIN 125-1 A A 5,3:27
- Placage:152 [Mate]: 1420-01-15 Coins superieur:3 ↔ DIN 125-1 A A 5,3:25
- Placage:153 [Mate]: 1420-01-15 Coins superieur:3 ↔ DIN 125-1 A A 5,3:26
- Placage:154 [Mate]: Vis à tête percée - Métrique M5x0,8 x 12:27 ↔ DIN 125-1 A A 5,3:28
- Affleurement:103 [Flush]: 1420-01-13 Noix M5:1 ↔ 1420-01-13 Noix M5:2
- Affleurement:104 [Flush]: 1420-01-13 Noix M5:1 ↔ 1420-01-13 Noix M5:3
- Affleurement:105 [Flush]: 1420-01-13 Noix M5:3 ↔ 1420-01-13 Noix M5:4
- Placage:155 [Mate]: Vis à tête percée - Métrique M5x0,8 x 12:42 ↔ 1420-01-13 Noix M5:3
- Placage:156 [Mate]: 1420-01-15 Coins superieur:1 ↔ 1420-01-13 Noix M5:1
- Placage:157 [Mate]: Vis à tête percée - Métrique M5x0,8 x 12:44 ↔ 1420-01-13 Noix M5:4
- Placage:158 [Mate]: Vis à tête percée - Métrique M5x0,8 x 12:43 ↔ 1420-01-13 Noix M5:2
- Placage:159 [Mate]: 1420-01-02 Profile horizontal 20x40x360:3 ↔ 1420-01-13 Noix M5:2
- Affleurement:106 [Flush]: 1420-01-13 Noix M5:1 ↔ 1420-01-13 Noix M5:3
- Affleurement:107 [Flush]: 1420-01-13 Noix M5:1 ↔ 1420-01-13 Noix M5:2
- Affleurement:108 [Flush]: 1420-01-13 Noix M5:2 ↔ 1420-01-13 Noix M5:4
- Affleurement:109 [Flush]: 1420-01-13 Noix M5:5 ↔ 1420-01-13 Noix M5:6
- Affleurement:110 [Flush]: 1420-01-13 Noix M5:6 ↔ 1420-01-13 Noix M5:7
- Affleurement:111 [Flush]: 1420-01-13 Noix M5:6 ↔ 1420-01-13 Noix M5:8
- Placage:160 [Mate]: Vis à tête percée - Métrique M5x0,8 x 12:34 ↔ 1420-01-13 Noix M5:6
- Placage:161 [Mate]: Vis à tête percée - Métrique M5x0,8 x 12:33 ↔ 1420-01-13 Noix M5:8
- Placage:162 [Mate]: Vis à tête percée - Métrique M5x0,8 x 12:36 ↔ 1420-01-13 Noix M5:7
- Placage:163 [Mate]: Vis à tête percée - Métrique M5x0,8 x 12:35 ↔ 1420-01-13 Noix M5:5
- Affleurement:112 [Flush]: 1420-01-13 Noix M5:1 ↔ 1420-01-13 Noix M5:7
- Affleurement:113 [Flush]: 1420-01-13 Noix M5:6 ↔ 1420-01-13 Noix M5:8
- Affleurement:114 [Flush]: 1420-01-13 Noix M5:5 ↔ 1420-01-13 Noix M5:8
- Affleurement:115 [Flush]: 1420-01-13 Noix M5:5 ↔ 1420-01-13 Noix M5:7
- Affleurement:116 [Flush]: 1420-01-13 Noix M5:9 ↔ 1420-01-13 Noix M5:10
- Affleurement:117 [Flush]: 1420-01-13 Noix M5:11 ↔ 1420-01-13 Noix M5:12
- Affleurement:118 [Flush]: 1420-01-13 Noix M5:10 ↔ 1420-01-13 Noix M5:11
- Placage:164 [Mate]: Vis à tête percée - Métrique M5x0,8 x 12:32 ↔ 1420-01-13 Noix M5:9
- Placage:165 [Mate]: Vis à tête percée - Métrique M5x0,8 x 12:31 ↔ 1420-01-13 Noix M5:10
- Placage:166 [Mate]: Vis à tête percée - Métrique M5x0,8 x 12:29 ↔ 1420-01-13 Noix M5:11
- Placage:167 [Mate]: Vis à tête percée - Métrique M5x0,8 x 12:30 ↔ 1420-01-13 Noix M5:12
- Affleurement:119 [Flush]: 1420-01-13 Noix M5:13 ↔ 1420-01-13 Noix M5:16
- Affleurement:120 [Flush]: 1420-01-13 Noix M5:13 ↔ 1420-01-13 Noix M5:14
- Affleurement:121 [Flush]: 1420-01-13 Noix M5:14 ↔ 1420-01-13 Noix M5:15
- Placage:168 [Mate]: Vis à tête percée - Métrique M5x0,8 x 12:28 ↔ 1420-01-13 Noix M5:13
- Placage:169 [Mate]: Vis à tête percée - Métrique M5x0,8 x 12:26 ↔ 1420-01-13 Noix M5:16
- Placage:170 [Mate]: Vis à tête percée - Métrique M5x0,8 x 12:25 ↔ 1420-01-13 Noix M5:14
- Placage:171 [Mate]: Vis à tête percée - Métrique M5x0,8 x 12:27 ↔ 1420-01-13 Noix M5:15
- Affleurement:122 [Flush]: 1420-01-13 Noix M5:13 ↔ 1420-01-13 Noix M5:16
- Affleurement:123 [Flush]: 1420-01-13 Noix M5:15 ↔ 1420-01-13 Noix M5:16
- Affleurement:124 [Flush]: 1420-01-13 Noix M5:14 ↔ 1420-01-13 Noix M5:15
- Placage:172 [Mate]: 1420-01-02 Profile horizontal 20x40x360:2 ↔ 1420-01-13 Noix M5:11
- Affleurement:125 [Flush]: 1420-01-13 Noix M5:11 ↔ 1420-01-13 Noix M5:16
- Affleurement:126 [Flush]: 1420-01-13 Noix M5:9 ↔ 1420-01-13 Noix M5:12
- Affleurement:127 [Flush]: 1420-01-13 Noix M5:11 ↔ 1420-01-13 Noix M5:12
- Affleurement:128 [Flush]: 1420-01-13 Noix M5:10 ↔ 1420-01-13 Noix M5:11
- Affleurement:129 [Flush]: 1420-01-13 Noix M5:18 ↔ 1420-01-13 Noix M5:19
- Affleurement:130 [Flush]: 1420-01-13 Noix M5:17 ↔ 1420-01-13 Noix M5:18
- Affleurement:131 [Flush]: 1420-01-13 Noix M5:18 ↔ 1420-01-13 Noix M5:20
- Placage:173 [Mate]: Vis à tête percée - Métrique M5x0,8 x 12:45 ↔ 1420-01-13 Noix M5:19
- Placage:174 [Mate]: Vis à tête percée - Métrique M5x0,8 x 12:46 ↔ 1420-01-13 Noix M5:20
- Placage:175 [Mate]: Vis à tête percée - Métrique M5x0,8 x 12:47 ↔ 1420-01-13 Noix M5:18
- Placage:176 [Mate]: Vis à tête percée - Métrique M5x0,8 x 12:49 ↔ 1420-01-13 Noix M5:17
- Affleurement:132 [Flush]: 1420-01-13 Noix M5:17 ↔ 1420-01-13 Noix M5:19
- Affleurement:133 [Flush]: 1420-01-13 Noix M5:18 ↔ 1420-01-13 Noix M5:20
- Affleurement:134 [Flush]: 1420-01-13 Noix M5:19 ↔ 1420-01-13 Noix M5:20
- Affleurement:135 [Flush]: 1420-01-13 Noix M5:22 ↔ 1420-01-13 Noix M5:23
- Affleurement:136 [Flush]: 1420-01-13 Noix M5:21 ↔ 1420-01-13 Noix M5:23
- Affleurement:137 [Flush]: 1420-01-13 Noix M5:21 ↔ 1420-01-13 Noix M5:24
- Placage:177 [Mate]: Vis à tête percée - Métrique M5x0,8 x 12:39 ↔ 1420-01-13 Noix M5:22
- Placage:178 [Mate]: Vis à tête percée - Métrique M5x0,8 x 12:38 ↔ 1420-01-13 Noix M5:23
- Placage:179 [Mate]: Vis à tête percée - Métrique M5x0,8 x 12:40 ↔ 1420-01-13 Noix M5:21
- Placage:180 [Mate]: Vis à tête percée - Métrique M5x0,8 x 12:37 ↔ 1420-01-13 Noix M5:24
- Affleurement:138 [Flush]: 1420-01-13 Noix M5:23 ↔ 1420-01-13 Noix M5:24
- Affleurement:139 [Flush]: 1420-01-13 Noix M5:21 ↔ 1420-01-13 Noix M5:22
- Affleurement:140 [Flush]: 1420-01-13 Noix M5:19 ↔ 1420-01-13 Noix M5:22
- Placage:181 [Mate]: 1420-01-02 Profile horizontal 20x40x360:1 ↔ 1420-01-13 Noix M5:18
- Affleurement:141 [Flush]: 1420-01-13 Noix M5:27 ↔ 1420-01-13 Noix M5:25
- Affleurement:142 [Flush]: 1420-01-13 Noix M5:28 ↔ 1420-01-13 Noix M5:26
- Affleurement:143 [Flush]: 1420-01-13 Noix M5:28 ↔ 1420-01-13 Noix M5:27
- Placage:182 [Mate]: 1420-01-13 Noix M5:25 ↔ Vis à tête percée - Métrique M5x0,8 x 12:23
- Placage:183 [Mate]: 1420-01-13 Noix M5:28 ↔ Vis à tête percée - Métrique M5x0,8 x 12:24
- Placage:184 [Mate]: 1420-01-13 Noix M5:26 ↔ Vis à tête percée - Métrique M5x0,8 x 12:21
- Placage:185 [Mate]: 1420-01-13 Noix M5:27 ↔ Vis à tête percée - Métrique M5x0,8 x 12:22